# Autodesk Inventor assembly: 主力车展开（运动仿真）
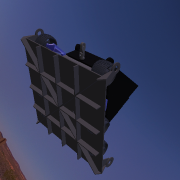
[picture p0: Inventor's stored thumbnail of the model, 180x180]
Saved by Autodesk Inventor 2012 (Build 160160000, 160)
## iProperties
Created: 2011-02-13
Part Number: 主力车展开（运动仿真）
Document SubType Name: Assembly
Designer: Administrator
Mass: 89839.9 g
Surface Area: 131223 cm^2
Volume: 68947.6 cm^3
Density: 1.30302 g/cm^3
Author: Administrator
## Documents named in this file (59)
- F:\探月车\湖北汽车工业学院 参赛作品\湖北汽车工业学院-动力先锋号\作品三维模型\主力车展开（运动仿真）.iam
- F:\探月车\湖北汽车工业学院 参赛作品\湖北汽车工业学院-动力先锋号\作品三维模型\中轮支撑.ipt
- F:\探月车\湖北汽车工业学院 参赛作品\湖北汽车工业学院-动力先锋号\作品三维模型\车轮.ipt
- F:\探月车\湖北汽车工业学院 参赛作品\湖北汽车工业学院-动力先锋号\作品三维模型\后轮支撑.ipt
- F:\探月车\湖北汽车工业学院 参赛作品\湖北汽车工业学院-动力先锋号\作品三维模型\后轮转向万向节(右).ipt
- F:\探月车\湖北汽车工业学院 参赛作品\湖北汽车工业学院-动力先锋号\作品三维模型\前轮支撑大臂.ipt
- F:\探月车\湖北汽车工业学院 参赛作品\湖北汽车工业学院-动力先锋号\作品三维模型\零件1.ipt
- F:\探月车\湖北汽车工业学院 参赛作品\湖北汽车工业学院-动力先锋号\作品三维模型\前轮支撑伸缩臂(右).ipt
- F:\探月车\湖北汽车工业学院 参赛作品\湖北汽车工业学院-动力先锋号\作品三维模型\前轮支撑大臂(左).ipt
- F:\探月车\湖北汽车工业学院 参赛作品\湖北汽车工业学院-动力先锋号\作品三维模型\前轮支撑伸缩臂(左).ipt
- F:\探月车\湖北汽车工业学院 参赛作品\湖北汽车工业学院-动力先锋号\作品三维模型\中轮支撑(左).ipt
- F:\探月车\湖北汽车工业学院 参赛作品\湖北汽车工业学院-动力先锋号\作品三维模型\后轮支撑(左).ipt
- F:\探月车\湖北汽车工业学院 参赛作品\湖北汽车工业学院-动力先锋号\作品三维模型\车轮转向万向节(左).ipt
- F:\探月车\湖北汽车工业学院 参赛作品\湖北汽车工业学院-动力先锋号\作品三维模型\车身下壳.ipt
- F:\探月车\湖北汽车工业学院 参赛作品\湖北汽车工业学院-动力先锋号\作品三维模型\正齿轮12.ipt
- F:\探月车\湖北汽车工业学院 参赛作品\湖北汽车工业学院-动力先锋号\作品三维模型\月球车\设计加速器\矩形花键联接2.iam
- F:\探月车\湖北汽车工业学院 参赛作品\湖北汽车工业学院-动力先锋号\作品三维模型\月球车\设计加速器\矩形花键联接3.iam
- F:\探月车\湖北汽车工业学院 参赛作品\湖北汽车工业学院-动力先锋号\作品三维模型\月球车\设计加速器\正齿轮21.ipt
- F:\探月车\湖北汽车工业学院 参赛作品\湖北汽车工业学院-动力先锋号\作品三维模型\月球车\设计加速器\锥齿轮11.ipt
- F:\探月车\湖北汽车工业学院 参赛作品\湖北汽车工业学院-动力先锋号\作品三维模型\月球车\设计加速器\锥齿轮21.ipt
- F:\探月车\湖北汽车工业学院 参赛作品\湖北汽车工业学院-动力先锋号\作品三维模型\月球车\设计加速器\正齿轮14.ipt
- F:\探月车\湖北汽车工业学院 参赛作品\湖北汽车工业学院-动力先锋号\作品三维模型\电池板-旋转式\1.ipt
- F:\探月车\湖北汽车工业学院 参赛作品\湖北汽车工业学院-动力先锋号\作品三维模型\电池板-旋转式\2.ipt
- F:\探月车\湖北汽车工业学院 参赛作品\湖北汽车工业学院-动力先锋号\作品三维模型\电池板-旋转式\3.ipt
- F:\探月车\湖北汽车工业学院 参赛作品\湖北汽车工业学院-动力先锋号\作品三维模型\电池板-旋转式\4.ipt
- F:\探月车\湖北汽车工业学院 参赛作品\湖北汽车工业学院-动力先锋号\作品三维模型\车身上盖.ipt
- F:\探月车\湖北汽车工业学院 参赛作品\湖北汽车工业学院-动力先锋号\作品三维模型\前臂拉杆.ipt
- F:\探月车\湖北汽车工业学院 参赛作品\湖北汽车工业学院-动力先锋号\作品三维模型\月球车\设计加速器\正齿轮23.ipt
- F:\探月车\湖北汽车工业学院 参赛作品\湖北汽车工业学院-动力先锋号\作品三维模型\摄像机架1.ipt
- F:\探月车\湖北汽车工业学院 参赛作品\湖北汽车工业学院-动力先锋号\作品三维模型\摄像机架蜗杆.ipt
- F:\探月车\湖北汽车工业学院 参赛作品\湖北汽车工业学院-动力先锋号\作品三维模型\摄像机架2.ipt
- F:\探月车\湖北汽车工业学院 参赛作品\湖北汽车工业学院-动力先锋号\作品三维模型\摄像头转轴.ipt
- F:\探月车\湖北汽车工业学院 参赛作品\湖北汽车工业学院-动力先锋号\作品三维模型\双目视觉摄像头.ipt
- F:\探月车\湖北汽车工业学院 参赛作品\湖北汽车工业学院-动力先锋号\作品三维模型\摄像头光圈1.ipt
- F:\探月车\湖北汽车工业学院 参赛作品\湖北汽车工业学院-动力先锋号\作品三维模型\摄像头光圈2.ipt
- F:\探月车\湖北汽车工业学院 参赛作品\湖北汽车工业学院-动力先锋号\作品三维模型\镜片1.ipt
- F:\探月车\湖北汽车工业学院 参赛作品\湖北汽车工业学院-动力先锋号\作品三维模型\机械臂大臂.ipt
- F:\探月车\湖北汽车工业学院 参赛作品\湖北汽车工业学院-动力先锋号\作品三维模型\机械臂中臂.ipt
- F:\探月车\湖北汽车工业学院 参赛作品\湖北汽车工业学院-动力先锋号\作品三维模型\机械臂小臂.ipt
- F:\探月车\湖北汽车工业学院 参赛作品\湖北汽车工业学院-动力先锋号\作品三维模型\小臂旋转关节.ipt
- F:\探月车\湖北汽车工业学院 参赛作品\湖北汽车工业学院-动力先锋号\作品三维模型\机械臂小臂2.ipt
- F:\探月车\湖北汽车工业学院 参赛作品\湖北汽车工业学院-动力先锋号\作品三维模型\机械手功能转盘.ipt
- F:\探月车\湖北汽车工业学院 参赛作品\湖北汽车工业学院-动力先锋号\作品三维模型\小型机械手大臂.ipt
- F:\探月车\湖北汽车工业学院 参赛作品\湖北汽车工业学院-动力先锋号\作品三维模型\小型机械手中臂.ipt
- F:\探月车\湖北汽车工业学院 参赛作品\湖北汽车工业学院-动力先锋号\作品三维模型\零件9.ipt
- F:\探月车\湖北汽车工业学院 参赛作品\湖北汽车工业学院-动力先锋号\作品三维模型\铲斗臂.ipt
- F:\探月车\湖北汽车工业学院 参赛作品\湖北汽车工业学院-动力先锋号\作品三维模型\光谱仪.ipt
- F:\探月车\湖北汽车工业学院 参赛作品\湖北汽车工业学院-动力先锋号\作品三维模型\小铣刀.ipt
- F:\探月车\湖北汽车工业学院 参赛作品\湖北汽车工业学院-动力先锋号\作品三维模型\探测棒.ipt
- F:\探月车\湖北汽车工业学院 参赛作品\湖北汽车工业学院-动力先锋号\作品三维模型\实验舱.ipt
- F:\探月车\湖北汽车工业学院 参赛作品\湖北汽车工业学院-动力先锋号\作品三维模型\实验舱门.ipt
- F:\探月车\湖北汽车工业学院 参赛作品\湖北汽车工业学院-动力先锋号\作品三维模型\中间车\天线.ipt
- F:\探月车\湖北汽车工业学院 参赛作品\湖北汽车工业学院-动力先锋号\作品三维模型\连接器1.ipt
- F:\探月车\湖北汽车工业学院 参赛作品\湖北汽车工业学院-动力先锋号\作品三维模型\连接器2.ipt
- F:\探月车\湖北汽车工业学院 参赛作品\湖北汽车工业学院-动力先锋号\作品三维模型\主力车卫星接收器.ipt
- F:\探月车\湖北汽车工业学院 参赛作品\湖北汽车工业学院-动力先锋号\作品三维模型\卫星接收器底座.ipt
- F:\探月车\湖北汽车工业学院 参赛作品\湖北汽车工业学院-动力先锋号\作品三维模型\箱盖.ipt
- F:\探月车\湖北汽车工业学院 参赛作品\湖北汽车工业学院-动力先锋号\作品三维模型\地面.ipt
- F:\探月车\湖北汽车工业学院 参赛作品\湖北汽车工业学院-动力先锋号\作品三维模型\卡扣.ipt
## Components (97 placed, 55 different names)
1. 矩形花键联接:2 [sub-assembly]
2. 矩形花键联接:3 [sub-assembly]
3. 连接器2:3 — 配合:323, 配合:324
4. 连接器1:3 — 配合:321, 配合:322, 配合:323, 配合:324
5. 箱盖:1 — 配合:325, 表面齐平:22, 表面齐平:23, 配合:326, 配合:327, 配合:328, 配合:329, 配合:330
6. 地面:1 — 配合:326
7. 卡扣:1 — 配合:329, 配合:330
8. 卡扣:2 — 配合:327, 配合:328
9. 中轮支撑:1 — 配合:5, 配合:6, 表面齐平:1, 配合:7, 配合:8, 配合:9
10. 后轮支撑:1 — 配合:3, 配合:4, 配合:5, 配合:6
11. 后轮转向万向节(右):1 — 配合:1, 配合:2, 配合:3, 配合:4
12. 前轮支撑大臂:1 — 表面齐平:1, 配合:7, 配合:35, 配合:36, 配合:43, 配合:44, 表面齐平:5, 配合:125, 配合:126, 配合:129, 配合:130
13. 车轮:1 — 配合:1, 配合:2
14. 车轮:2 — 配合:8, 配合:9
15. 零件1:1 — 配合:125, 配合:126, 配合:131, 配合:132
16. 前轮支撑伸缩臂(右):1 — 配合:14, 配合:15, 配合:127, 配合:128, 配合:131, 配合:132
17. 后轮转向万向节(右):2 — 配合:14, 配合:15, 配合:16, 配合:17
18. 车轮:3 — 配合:16, 配合:17
19. 前轮支撑大臂(左):1 — 配合:24, 表面齐平:2, 配合:37, 配合:38, 配合:45, 配合:46, 表面齐平:6, 配合:134, 配合:137, 配合:138, 配合:141
20. 零件1:2 — 配合:134, 配合:139, 配合:140, 配合:141
21. 前轮支撑伸缩臂(左):1 — 配合:27, 配合:28, 配合:135, 配合:136, 配合:139, 配合:140
22. 中轮支撑(左):1 — 配合:22, 配合:23, 配合:24, 表面齐平:2, 配合:30, 配合:33
23. 后轮支撑(左):1 — 配合:22, 配合:23, 配合:25, 配合:26
24. 车轮转向万向节(左):1 — 配合:25, 配合:26, 配合:31, 配合:32
25. 车轮转向万向节(左):2 — 配合:27, 配合:28, 配合:29, 配合:34
26. 车轮:4 — 配合:29, 配合:34
27. 车轮:5 — 配合:30, 配合:33
28. 车轮:6 — 配合:31, 配合:32
29. 车身下壳:1 — 配合:35, 配合:36, 配合:37, 配合:38, 配合:55, 配合:56, 配合:57, 配合:58, 配合:68, 表面齐平:10, 配合:142, 表面齐平:17, 配合:166, 配合:167, 配合:191, 表面齐平:20, 表面齐平:21, 配合:301, 配合:302, 配合:321, 配合:322
30. 正齿轮1:1 — 配合:43, 配合:44, 表面齐平:5
31. 正齿轮1:2 — 配合:45, 配合:46, 表面齐平:6
32. 正齿轮2:1 — 配合:52, 配合:53, 配合:54, 配合:55, 配合:56
33. 正齿轮2:2 — 配合:49, 配合:50, 配合:51, 配合:57, 配合:58
34. 锥齿轮1:1 — 配合:59, 配合:60
35. 锥齿轮2:1 — 配合:49, 配合:50, 配合:51
36. 锥齿轮2:2 — 配合:52, 配合:53, 配合:54
37. 正齿轮1:3 — 配合:59, 配合:60, 配合:61, 配合:62, 配合:63, 配合:64, 配合:68, 表面齐平:10
38. 锥齿轮1:2 — 配合:63, 配合:64
39. 锥齿轮1:3 — 配合:61, 配合:62
40. 1:1 — 配合:123, 表面齐平:15
41. 2:1
42. 3:1
43. 3:2
44. 3:3
45. 4:1 — 配合:123, 表面齐平:15, 配合:124, 表面齐平:16
46. 车身上盖:1 — 配合:143, 配合:144, 配合:295, 配合:296, 配合:319, 配合:320
47. 4:2 — 配合:121, 表面齐平:13, 配合:122, 表面齐平:14
48. 3:4
49. 3:5
50. 3:6
51. 2:3
52. 1:3 — 配合:124, 表面齐平:16
53. 3:7
54. 3:8
55. 3:9
56. 2:4
57. 1:4 — 配合:121, 表面齐平:13
58. 3:10 — 配合:118
59. 3:11 — 配合:117, 配合:118
60. 3:12 — 配合:116, 配合:117
61. 1:2 — 配合:115, 配合:122, 表面齐平:14
62. 2:2 — 配合:115, 配合:116
63. 前臂拉杆:1 — 配合:127, 配合:128, 配合:129, 配合:130
64. 前臂拉杆:2 — 配合:135, 配合:136, 配合:137, 配合:138
65. 正齿轮2:3 — 配合:142, 表面齐平:17
66. 摄像机架1:1 — 配合:143, 配合:144, 配合:145, 配合:146, 配合:148, 配合:149
67. 摄像机架蜗杆:1 — 配合:145, 配合:146, 配合:147
68. 摄像机架2:1 — 配合:147, 配合:148, 配合:149, 配合:150, 配合:163
69. 摄像头转轴:1 — 配合:150, 配合:152, 配合:153, 配合:163
70. 双目视觉摄像头:1 — 配合:152, 配合:153, 配合:158, 配合:162
71. 摄像头光圈1:1 — 配合:156, 配合:158
72. 摄像头光圈2:1 — 配合:154, 配合:156, 配合:165
73. 镜片1:1 — 配合:154, 配合:165
74. 摄像头光圈1:2 — 配合:161, 配合:162
75. 摄像头光圈2:2 — 配合:159, 配合:161, 配合:164
76. 镜片1:2 — 配合:159, 配合:164
77. 机械臂大臂:1 — 配合:166, 配合:167, 配合:168, 配合:169
78. 机械臂中臂:1 — 配合:168, 配合:169, 配合:174, 配合:175
79. 机械臂小臂:1 — 配合:172, 配合:173, 配合:176, 配合:177
80. 小臂旋转关节:1 — 配合:172, 配合:173, 配合:178, 配合:179
81. 机械臂小臂2:1 — 配合:174, 配合:175, 配合:176, 配合:177
82. 机械手功能转盘:1 — 配合:178, 配合:179, 配合:180, 表面齐平:18, 配合:181, 配合:182, 配合:188, 配合:189, 配合:190
83. 镜片1:3 — 配合:180, 表面齐平:18
84. 小型机械手大臂:1 — 配合:181, 配合:182, 配合:183, 表面齐平:19
85. 小型机械手中臂:1 — 配合:183, 表面齐平:19, 配合:186, 配合:187
86. 零件9:1 — 配合:184, 配合:185
87. 铲斗臂:1 — 配合:184, 配合:185, 配合:186, 配合:187
88. 光谱仪:1 — 配合:188
89. 小铣刀:1 — 配合:189
90. 探测棒:1 — 配合:190
91. 实验舱:1 — 配合:191, 表面齐平:20, 表面齐平:21, 配合:192, 配合:193
92. 实验舱门:1 — 配合:192, 配合:193
93. 天线:2 — 配合:295, 配合:296
94. 连接器1:2 — 配合:301, 配合:302, 配合:305, 配合:306
95. 连接器2:2 — 配合:305, 配合:306
96. 主力车卫星接收器:1 — 配合:317, 配合:318
97. 卫星接收器底座:1 — 配合:317, 配合:318, 配合:319, 配合:320
## Relationships (192: Mate 174, Flush 18)
- 配合:1 [Mate]: 后轮转向万向节(右):1 ↔ 车轮:1
- 配合:2 [Mate]: 后轮转向万向节(右):1 ↔ 车轮:1
- 配合:3 [Mate]: 后轮支撑:1 ↔ 后轮转向万向节(右):1
- 配合:4 [Mate]: 后轮支撑:1 ↔ 后轮转向万向节(右):1
- 配合:5 [Mate]: 中轮支撑:1 ↔ 后轮支撑:1
- 配合:6 [Mate]: 中轮支撑:1 ↔ 后轮支撑:1
- 表面齐平:1 [Flush]: 中轮支撑:1 ↔ 前轮支撑大臂:1
- 配合:7 [Mate]: 中轮支撑:1 ↔ 前轮支撑大臂:1
- 配合:8 [Mate]: 中轮支撑:1 ↔ 车轮:2
- 配合:9 [Mate]: 中轮支撑:1 ↔ 车轮:2
- 配合:14 [Mate]: 前轮支撑伸缩臂(右):1 ↔ 后轮转向万向节(右):2
- 配合:15 [Mate]: 前轮支撑伸缩臂(右):1 ↔ 后轮转向万向节(右):2
- 配合:16 [Mate]: 后轮转向万向节(右):2 ↔ 车轮:3
- 配合:17 [Mate]: 后轮转向万向节(右):2 ↔ 车轮:3
- 配合:22 [Mate]: 中轮支撑(左):1 ↔ 后轮支撑(左):1
- 配合:23 [Mate]: 中轮支撑(左):1 ↔ 后轮支撑(左):1
- 配合:24 [Mate]: 前轮支撑大臂(左):1 ↔ 中轮支撑(左):1
- 表面齐平:2 [Flush]: 前轮支撑大臂(左):1 ↔ 中轮支撑(左):1
- 配合:25 [Mate]: 后轮支撑(左):1 ↔ 车轮转向万向节(左):1
- 配合:26 [Mate]: 后轮支撑(左):1 ↔ 车轮转向万向节(左):1
- 配合:27 [Mate]: 前轮支撑伸缩臂(左):1 ↔ 车轮转向万向节(左):2
- 配合:28 [Mate]: 前轮支撑伸缩臂(左):1 ↔ 车轮转向万向节(左):2
- 配合:29 [Mate]: 车轮转向万向节(左):2 ↔ 车轮:4
- 配合:30 [Mate]: 中轮支撑(左):1 ↔ 车轮:5
- 配合:31 [Mate]: 车轮转向万向节(左):1 ↔ 车轮:6
- 配合:32 [Mate]: 车轮转向万向节(左):1 ↔ 车轮:6
- 配合:33 [Mate]: 中轮支撑(左):1 ↔ 车轮:5
- 配合:34 [Mate]: 车轮转向万向节(左):2 ↔ 车轮:4
- 配合:35 [Mate]: 前轮支撑大臂:1 ↔ 车身下壳:1
- 配合:36 [Mate]: 前轮支撑大臂:1 ↔ 车身下壳:1
- 配合:37 [Mate]: 前轮支撑大臂(左):1 ↔ 车身下壳:1
- 配合:38 [Mate]: 前轮支撑大臂(左):1 ↔ 车身下壳:1
- 配合:43 [Mate]: 前轮支撑大臂:1 ↔ 正齿轮1:1
- 配合:44 [Mate]: 前轮支撑大臂:1 ↔ 正齿轮1:1
- 表面齐平:5 [Flush]: 前轮支撑大臂:1 ↔ 正齿轮1:1
- 配合:45 [Mate]: 前轮支撑大臂(左):1 ↔ 正齿轮1:2
- 配合:46 [Mate]: 前轮支撑大臂(左):1 ↔ 正齿轮1:2
- 表面齐平:6 [Flush]: 前轮支撑大臂(左):1 ↔ 正齿轮1:2
- 配合:49 [Mate]: 正齿轮2:2 ↔ 锥齿轮2:1
- 配合:50 [Mate]: 正齿轮2:2 ↔ 锥齿轮2:1
- 配合:51 [Mate]: 正齿轮2:2 ↔ 锥齿轮2:1
- 配合:52 [Mate]: 正齿轮2:1 ↔ 锥齿轮2:2
- 配合:53 [Mate]: 正齿轮2:1 ↔ 锥齿轮2:2
- 配合:54 [Mate]: 正齿轮2:1 ↔ 锥齿轮2:2
- 配合:55 [Mate]: 车身下壳:1 ↔ 正齿轮2:1
- 配合:56 [Mate]: 车身下壳:1 ↔ 正齿轮2:1
- 配合:57 [Mate]: 车身下壳:1 ↔ 正齿轮2:2
- 配合:58 [Mate]: 车身下壳:1 ↔ 正齿轮2:2
- 配合:59 [Mate]: 锥齿轮1:1 ↔ 正齿轮1:3
- 配合:60 [Mate]: 锥齿轮1:1 ↔ 正齿轮1:3
- 配合:61 [Mate]: 正齿轮1:3 ↔ 锥齿轮1:3
- 配合:62 [Mate]: 正齿轮1:3 ↔ 锥齿轮1:3
- 配合:63 [Mate]: 正齿轮1:3 ↔ 锥齿轮1:2
- 配合:64 [Mate]: 正齿轮1:3 ↔ 锥齿轮1:2
- 配合:68 [Mate]: 车身下壳:1 ↔ 正齿轮1:3
- 表面齐平:10 [Flush]: 车身下壳:1 ↔ 正齿轮1:3
- [Flush]: 车身下壳:1 ↔ 车身上盖:1
- [Flush]: 车身下壳:1 ↔ 车身上盖:1
- [Mate]: 车身下壳:1 ↔ 车身上盖:1
- [Mate]: 3:2 ↔ 3:3
- [Mate]: 3:1 ↔ 3:2
- [Mate]: 3:1 ↔ 3:2
- [Mate]: 3:2 ↔ 3:3
- [Mate]: 2:1 ↔ 3:3
- [Mate]: 1:1 ↔ 2:1
- [Mate]: 2:1 ↔ 3:3
- [Mate]: 1:1 ↔ 2:1
- [Mate]: 4:1 ↔ 车身上盖:1
- [Mate]: 4:1 ↔ 车身上盖:1
- [Mate]: 车身上盖:1 ↔ 4:2
- [Mate]: 车身上盖:1 ↔ 4:2
- [Mate]: 3:4 ↔ 3:5
- [Mate]: 3:4 ↔ 3:6
- [Mate]: 3:4 ↔ 3:6
- [Mate]: 3:4 ↔ 3:5
- [Mate]: 3:6 ↔ 2:3
- [Mate]: 3:6 ↔ 2:3
- [Mate]: 2:3 ↔ 1:3
- [Mate]: 2:3 ↔ 1:3
- [Mate]: 3:8 ↔ 3:9
- [Mate]: 3:7 ↔ 3:9
- [Mate]: 3:8 ↔ 3:9
- [Mate]: 3:7 ↔ 3:9
- [Mate]: 3:7 ↔ 2:4
- [Mate]: 3:7 ↔ 2:4
- [Mate]: 2:4 ↔ 1:4
- [Mate]: 2:4 ↔ 1:4
- [Mate]: 3:10 ↔ 3:11
- [Mate]: 3:11 ↔ 3:12
- [Mate]: 3:12 ↔ 2:2
- [Mate]: 1:2 ↔ 2:2
- 配合:115 [Mate]: 1:2 ↔ 2:2
- 配合:116 [Mate]: 3:12 ↔ 2:2
- 配合:117 [Mate]: 3:11 ↔ 3:12
- 配合:118 [Mate]: 3:10 ↔ 3:11
- 配合:121 [Mate]: 4:2 ↔ 1:4
- 表面齐平:13 [Flush]: 4:2 ↔ 1:4
- 配合:122 [Mate]: 4:2 ↔ 1:2
- 表面齐平:14 [Flush]: 4:2 ↔ 1:2
- 配合:123 [Mate]: 1:1 ↔ 4:1
- 表面齐平:15 [Flush]: 1:1 ↔ 4:1
- 配合:124 [Mate]: 4:1 ↔ 1:3
- 表面齐平:16 [Flush]: 4:1 ↔ 1:3
- 配合:125 [Mate]: 前轮支撑大臂:1 ↔ 零件1:1
- 配合:126 [Mate]: 前轮支撑大臂:1 ↔ 零件1:1
- 配合:127 [Mate]: 前轮支撑伸缩臂(右):1 ↔ 前臂拉杆:1
- 配合:128 [Mate]: 前轮支撑伸缩臂(右):1 ↔ 前臂拉杆:1
- 配合:129 [Mate]: 前轮支撑大臂:1 ↔ 前臂拉杆:1
- 配合:130 [Mate]: 前轮支撑大臂:1 ↔ 前臂拉杆:1
- 配合:131 [Mate]: 零件1:1 ↔ 前轮支撑伸缩臂(右):1
- 配合:132 [Mate]: 零件1:1 ↔ 前轮支撑伸缩臂(右):1
- 配合:134 [Mate]: 前轮支撑大臂(左):1 ↔ 零件1:2
- 配合:135 [Mate]: 前轮支撑伸缩臂(左):1 ↔ 前臂拉杆:2
- 配合:136 [Mate]: 前轮支撑伸缩臂(左):1 ↔ 前臂拉杆:2
- 配合:137 [Mate]: 前轮支撑大臂(左):1 ↔ 前臂拉杆:2
- 配合:138 [Mate]: 前轮支撑大臂(左):1 ↔ 前臂拉杆:2
- 配合:139 [Mate]: 零件1:2 ↔ 前轮支撑伸缩臂(左):1
- 配合:140 [Mate]: 零件1:2 ↔ 前轮支撑伸缩臂(左):1
- 配合:141 [Mate]: 前轮支撑大臂(左):1 ↔ 零件1:2
- 配合:142 [Mate]: 车身下壳:1 ↔ 正齿轮2:3
- 表面齐平:17 [Flush]: 车身下壳:1 ↔ 正齿轮2:3
- 配合:143 [Mate]: 车身上盖:1 ↔ 摄像机架1:1
- 配合:144 [Mate]: 车身上盖:1 ↔ 摄像机架1:1
- 配合:145 [Mate]: 摄像机架1:1 ↔ 摄像机架蜗杆:1
- 配合:146 [Mate]: 摄像机架1:1 ↔ 摄像机架蜗杆:1
- 配合:147 [Mate]: 摄像机架蜗杆:1 ↔ 摄像机架2:1
- 配合:148 [Mate]: 摄像机架1:1 ↔ 摄像机架2:1
- 配合:149 [Mate]: 摄像机架1:1 ↔ 摄像机架2:1
- 配合:150 [Mate]: 摄像机架2:1 ↔ 摄像头转轴:1
- 配合:152 [Mate]: 摄像头转轴:1 ↔ 双目视觉摄像头:1
- 配合:153 [Mate]: 摄像头转轴:1 ↔ 双目视觉摄像头:1
- 配合:154 [Mate]: 摄像头光圈2:1 ↔ 镜片1:1
- 配合:156 [Mate]: 摄像头光圈1:1 ↔ 摄像头光圈2:1
- 配合:158 [Mate]: 双目视觉摄像头:1 ↔ 摄像头光圈1:1
- 配合:159 [Mate]: 摄像头光圈2:2 ↔ 镜片1:2
- 配合:161 [Mate]: 摄像头光圈1:2 ↔ 摄像头光圈2:2
- 配合:162 [Mate]: 双目视觉摄像头:1 ↔ 摄像头光圈1:2
- 配合:163 [Mate]: 摄像机架2:1 ↔ 摄像头转轴:1
- 配合:164 [Mate]: 摄像头光圈2:2 ↔ 镜片1:2
- 配合:165 [Mate]: 摄像头光圈2:1 ↔ 镜片1:1
- 配合:166 [Mate]: 车身下壳:1 ↔ 机械臂大臂:1
- 配合:167 [Mate]: 车身下壳:1 ↔ 机械臂大臂:1
- 配合:168 [Mate]: 机械臂大臂:1 ↔ 机械臂中臂:1
- 配合:169 [Mate]: 机械臂大臂:1 ↔ 机械臂中臂:1
- 配合:172 [Mate]: 机械臂小臂:1 ↔ 小臂旋转关节:1
- 配合:173 [Mate]: 机械臂小臂:1 ↔ 小臂旋转关节:1
- 配合:174 [Mate]: 机械臂中臂:1 ↔ 机械臂小臂2:1
- 配合:175 [Mate]: 机械臂中臂:1 ↔ 机械臂小臂2:1
- 配合:176 [Mate]: 机械臂小臂:1 ↔ 机械臂小臂2:1
- 配合:177 [Mate]: 机械臂小臂:1 ↔ 机械臂小臂2:1
- 配合:178 [Mate]: 小臂旋转关节:1 ↔ 机械手功能转盘:1
- 配合:179 [Mate]: 小臂旋转关节:1 ↔ 机械手功能转盘:1
- 配合:180 [Mate]: 机械手功能转盘:1 ↔ 镜片1:3
- 表面齐平:18 [Flush]: 机械手功能转盘:1 ↔ 镜片1:3
- 配合:181 [Mate]: 机械手功能转盘:1 ↔ 小型机械手大臂:1
- 配合:182 [Mate]: 机械手功能转盘:1 ↔ 小型机械手大臂:1
- 配合:183 [Mate]: 小型机械手大臂:1 ↔ 小型机械手中臂:1
- 表面齐平:19 [Flush]: 小型机械手大臂:1 ↔ 小型机械手中臂:1
- 配合:184 [Mate]: 零件9:1 ↔ 铲斗臂:1
- 配合:185 [Mate]: 零件9:1 ↔ 铲斗臂:1
- 配合:186 [Mate]: 小型机械手中臂:1 ↔ 铲斗臂:1
- 配合:187 [Mate]: 小型机械手中臂:1 ↔ 铲斗臂:1
- 配合:188 [Mate]: 机械手功能转盘:1 ↔ 光谱仪:1
- 配合:189 [Mate]: 机械手功能转盘:1 ↔ 小铣刀:1
- 配合:190 [Mate]: 机械手功能转盘:1 ↔ 探测棒:1
- 配合:191 [Mate]: 车身下壳:1 ↔ 实验舱:1
- 表面齐平:20 [Flush]: 车身下壳:1 ↔ 实验舱:1
- 表面齐平:21 [Flush]: 车身下壳:1 ↔ 实验舱:1
- 配合:192 [Mate]: 实验舱:1 ↔ 实验舱门:1
- 配合:193 [Mate]: 实验舱:1 ↔ 实验舱门:1
- 配合:295 [Mate]: 车身上盖:1 ↔ 天线:2
- 配合:296 [Mate]: 车身上盖:1 ↔ 天线:2
- 配合:301 [Mate]: 车身下壳:1 ↔ 连接器1:2
- 配合:302 [Mate]: 车身下壳:1 ↔ 连接器1:2
- 配合:305 [Mate]: 连接器1:2 ↔ 连接器2:2
- 配合:306 [Mate]: 连接器1:2 ↔ 连接器2:2
- 配合:317 [Mate]: 主力车卫星接收器:1 ↔ 卫星接收器底座:1
- 配合:318 [Mate]: 主力车卫星接收器:1 ↔ 卫星接收器底座:1
- 配合:319 [Mate]: 车身上盖:1 ↔ 卫星接收器底座:1
- 配合:320 [Mate]: 车身上盖:1 ↔ 卫星接收器底座:1
- 配合:321 [Mate]: 连接器1:3 ↔ 车身下壳:1
- 配合:322 [Mate]: 连接器1:3 ↔ 车身下壳:1
- 配合:323 [Mate]: 连接器2:3 ↔ 连接器1:3
- 配合:324 [Mate]: 连接器2:3 ↔ 连接器1:3
- 配合:325 [Mate]: 箱盖:1
- 表面齐平:22 [Flush]: 箱盖:1
- 表面齐平:23 [Flush]: 箱盖:1
- 配合:326 [Mate]: 箱盖:1 ↔ 地面:1
- 配合:327 [Mate]: 箱盖:1 ↔ 卡扣:2
- 配合:328 [Mate]: 箱盖:1 ↔ 卡扣:2
- 配合:329 [Mate]: 箱盖:1 ↔ 卡扣:1
- 配合:330 [Mate]: 箱盖:1 ↔ 卡扣:1
## Named parameters: d139_d0 = 0 mm, d140_d1 = 0 mm, d141_d2 = 0 mm, d142_d3 = 0 mm, d143_d4 = 0 mm, d144_d5 = 0 mm, d150_d6 = 0 mm, d151_d7 = 0 mm, d156_d14 = 0 mm, d157_d15 = 0 mm, d161_d19 = 0 mm, d169_d44 = 0 mm, d170_d46 = 0 mm, d171_d22 = 0 mm, d172_d23 = 0 mm, d173_d24 = 0 mm, d174_d25 = 0 mm, d175_d26 = 0 mm, d176_d27 = 0 mm, d177_d28 = 0 mm, d178_d29 = 0 mm, d179_d30 = 0 mm, d180_d31 = 0 mm, d181_d32 = 0 mm, Simulation_Timeline = 19.1406
